# Autodesk Inventor assembly: robot pierwszy
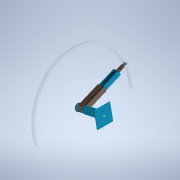
[picture p0: Inventor's stored thumbnail of the model, 180x180]
Saved by Autodesk Inventor 2022 (Build 260153000, 153)
## iProperties
Created: 2022-06-14
Part Number: robot pierwszy
Document SubType Name: Assembly
Designer: admin
Author: admin
## Documents named in this file (7)
- C:\Users\admin\Dropbox\semestr 4\Modelowanie i sterowanie robotów\laboratoria\projekcik\robot pierwszy.iam
- C:\Users\admin\Dropbox\semestr 4\Modelowanie i sterowanie robotów\laboratoria\projekcik\1przegub.ipt
- C:\Users\admin\Dropbox\semestr 4\Modelowanie i sterowanie robotów\laboratoria\projekcik\czesc2.ipt
- C:\Users\admin\Dropbox\semestr 4\Modelowanie i sterowanie robotów\laboratoria\projekcik\czesc3.ipt
- C:\Users\admin\Dropbox\semestr 4\Modelowanie i sterowanie robotów\laboratoria\projekcik\czesc5.ipt
- C:\Users\admin\Dropbox\semestr 4\Modelowanie i sterowanie robotów\laboratoria\projekcik\Część6.ipt
- C:\Users\admin\Dropbox\semestr 4\Modelowanie i sterowanie robotów\laboratoria\projekcik\przestrzeń robocza.ipt
## Components (7 placed, 6 different names)
1. 1przegub:1 — Zestawiające:2, Zestawiające:5, Zestawiające:7, Zestawiające:8, Zestawiające:11
2. czesc2:1 — Zestawiające:2, przesuwne:1, Zestawiające:6, Zestawiające:9
3. czesc3:1 — przesuwne:1, Zestawiające:3, Zestawiające:4
4. czesc5:1 — Zestawiające:3, Zestawiające:4, Równoległe:1
5. Część6:1 — Zestawiające:5, Zestawiające:6
6. Część6:2 — Zestawiające:7, Zestawiające:8, Zestawiające:9
7. przestrzeń robocza:1 — Zestawiające:10, Równoległe:1
## Relationships (12: Mate 10, TranslationJoint 1, Flush 1)
- Zestawiające:2 [Mate]: 1przegub:1 ↔ czesc2:1
- przesuwne:1 [TranslationJoint]: czesc2:1 ↔ czesc3:1
- Zestawiające:3 [Mate]: czesc3:1 ↔ czesc5:1
- Zestawiające:4 [Mate]: czesc3:1 ↔ czesc5:1
- Zestawiające:5 [Mate]: 1przegub:1 ↔ Część6:1
- Zestawiające:6 [Mate]: czesc2:1 ↔ Część6:1
- Zestawiające:7 [Mate]: 1przegub:1 ↔ Część6:2
- Zestawiające:8 [Mate]: 1przegub:1 ↔ Część6:2
- Zestawiające:9 [Mate]: czesc2:1 ↔ Część6:2
- Zestawiające:10 [Mate]: przestrzeń robocza:1
- Zestawiające:11 [Mate]: 1przegub:1
- Równoległe:1 [Flush]: czesc5:1 ↔ przestrzeń robocza:1
